# Autodesk Inventor assembly: CJ2B10-124Z(0_1_0)
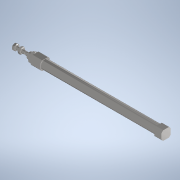
[picture p0: Inventor's stored thumbnail of the model, 180x180]
Saved by Autodesk Inventor 2022.3 (Build 263350000, 350)
## iProperties
Created: 2020-02-10
Part Number: CJ2B10-124Z(0_1_0)
Description: STEP AP203
Document SubType Name: Assembly
Designer: Hagihara Yuya
Sending System: PARTsolutions
Title: p:/temp/worker_6/temp/exporttempdir_3952_1651_Dq4ul/format_0/CJ2B10-124Z(0_1_0).stp
Revision Number: NONE
## Documents named in this file (5)
- C:\Users\YusukeKunita\Documents\GrabCAD\Development\BasicParts\AirCylinder\CJ2B10-124Z\CJ2B10-124Z.iam
- C:\Users\YusukeKunita\Documents\GrabCAD\Development\BasicParts\AirCylinder\CJ2B10-124Z\CJ2B10-124Z_BODY.ipt
- C:\Users\YusukeKunita\Documents\GrabCAD\Development\BasicParts\AirCylinder\CJ2B10-124Z\CJ2B10-124Z_ROD.ipt
- C:\Users\YusukeKunita\Documents\GrabCAD\Development\BasicParts\AirCylinder\CJ2B10-124Z\NTJ-010C.ipt
- C:\Users\YusukeKunita\Documents\GrabCAD\Development\BasicParts\AirCylinder\CJ2B10-124Z\SNJ-010C.ipt
## Components (5 placed, 5 different names)
1. NAUO1 — 円柱状:1, 円柱状:2
2. NAUO2 — 円柱状:1, 回転:1
3. NAUO3 — 回転:1, 円柱状:3
4. NAUO4 — 円柱状:3
5. NAUO5 — 円柱状:2
## Relationships (4: CylindricalJoint 3, RevoluteJoint 1)
- 円柱状:1 [CylindricalJoint]: NAUO1 ↔ NAUO2
- 円柱状:2 [CylindricalJoint]: NAUO1 ↔ NAUO5
- 回転:1 [RevoluteJoint] (-8 mm): NAUO2 ↔ NAUO3
- 円柱状:3 [CylindricalJoint]: NAUO3 ↔ NAUO4
